# Autodesk Inventor assembly: 組合1
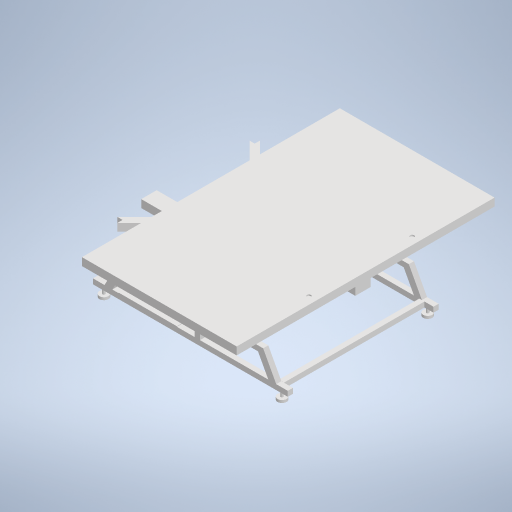
[picture p0: Inventor's stored thumbnail of the model, 512x512]
Saved by Autodesk Inventor 2024 (Build 280153000, 153)
## iProperties
Created: 2024-10-15
Part Number: 組合1
Document SubType Name: Assembly
Designer: jerry
Author: jerry
## Documents named in this file (12)
- C:\Users\jerry\Desktop\Inventor Model\組合1.iam
- C:\Users\jerry\Desktop\Inventor Model\Body Actuator.ipt
- C:\Users\jerry\Desktop\Inventor Model\DOF1.ipt
- C:\Users\jerry\Desktop\Inventor Model\DOF2.ipt
- C:\Users\jerry\Desktop\Inventor Model\DOF3.ipt
- C:\Users\jerry\Desktop\Inventor Model\DOF4.ipt
- C:\Users\jerry\Desktop\Inventor Model\DOF5.ipt
- C:\Users\jerry\Desktop\Inventor Model\DOF6.ipt
- C:\Users\jerry\Desktop\Inventor Model\DOF7.ipt
- C:\Users\jerry\Desktop\Inventor Model\DOF8.ipt
- C:\Users\jerry\Desktop\Inventor Model\DOF9.ipt
- C:\Users\jerry\Desktop\Inventor Model\DOF10.ipt
## Components (11 placed, 11 different names)
1. Body Actuator:1 — 齊平:1, 齊平:3
2. DOF1:1 — 齊平:1, 齊平:2
3. DOF2:1 — 齊平:2, 齊平:4, 齊平:6
4. DOF3:1 — 齊平:3
5. DOF4:1 — 齊平:4, 齊平:5
6. DOF5:1 — 齊平:5, 齊平:7, 齊平:8
7. DOF6:1 — 齊平:6
8. DOF7:1 — 齊平:7, 齊平:10
9. DOF8:1 — 齊平:8, 齊平:9
10. DOF9:1 — 齊平:9
11. DOF10:1 — 齊平:10
## Relationships (10: Flush 10)
- 齊平:1 [Flush]: Body Actuator:1 ↔ DOF1:1
- 齊平:2 [Flush]: DOF1:1 ↔ DOF2:1
- 齊平:3 [Flush]: Body Actuator:1 ↔ DOF3:1
- 齊平:4 [Flush]: DOF2:1 ↔ DOF4:1
- 齊平:5 [Flush]: DOF4:1 ↔ DOF5:1
- 齊平:6 [Flush]: DOF2:1 ↔ DOF6:1
- 齊平:7 [Flush]: DOF5:1 ↔ DOF7:1
- 齊平:8 [Flush]: DOF5:1 ↔ DOF8:1
- 齊平:9 [Flush]: DOF8:1 ↔ DOF9:1
- 齊平:10 [Flush]: DOF7:1 ↔ DOF10:1
